# Autodesk Inventor assembly: New Ripstik Assembly
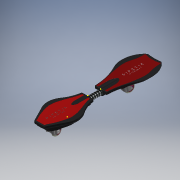
[picture p0: Inventor's stored thumbnail of the model, 180x180]
Saved by Autodesk Inventor 2018 (Build 220112000, 112)
## iProperties
Created: 2018-04-07
Part Number: New Ripstik Assembly
Document SubType Name: Assembly
Designer: Cole
Author: Cole
## Documents named in this file (7)
- P:\IED\SchoolCAD\ReverseEngineering\New Ripstik Assembly.iam
- P:\IED\SchoolCAD\ReverseEngineering\Back Board Assembly.iam
- P:\IED\SchoolCAD\ReverseEngineering\Front Board Assembly.iam
- P:\IED\SchoolCAD\ReverseEngineering\Rotation Resistor Assembly.iam
- P:\IED\SchoolCAD\ReverseEngineering\Middle Rod Assembly.iam
- P:\IED\SchoolCAD\ReverseEngineering\Wheel-Axel Assembly.iam
- P:\IED\SchoolCAD\ReverseEngineering\Double Sided Bolt Assembly.iam
## Components (8 placed, 6 different names)
1. Back Board Assembly:1 [sub-assembly] — Insert:2, Insert:8
2. Front Board Assembly:1 [sub-assembly] — Insert:1, Insert:3, Insert:6
3. Rotation Resistor Assembly:1 [sub-assembly] — Insert:3
4. Middle Rod Assembly:1 [sub-assembly] — Insert:1, Insert:2
5. Wheel-Axel Assembly:1 [sub-assembly] — Insert:7
6. Wheel-Axel Assembly:2 [sub-assembly] — Insert:9
7. Double Sided Bolt Assembly:1 [sub-assembly] — Insert:6, Insert:7
8. Double Sided Bolt Assembly:2 [sub-assembly] — Insert:8, Insert:9
## Relationships (7: Insert 7)
- Insert:1: Front Board Assembly:1 ↔ Middle Rod Assembly:1
- Insert:2: Back Board Assembly:1 ↔ Middle Rod Assembly:1
- Insert:3 (25.4 mm): Front Board Assembly:1 ↔ Rotation Resistor Assembly:1
- Insert:6: Front Board Assembly:1 ↔ Double Sided Bolt Assembly:1
- Insert:7: Wheel-Axel Assembly:1 ↔ Double Sided Bolt Assembly:1
- Insert:8: Back Board Assembly:1 ↔ Double Sided Bolt Assembly:2
- Insert:9: Wheel-Axel Assembly:2 ↔ Double Sided Bolt Assembly:2
